# Autodesk Inventor assembly: partial assembly
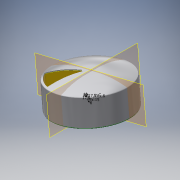
[picture p0: Inventor's stored thumbnail of the model, 180x180]
Saved by Autodesk Inventor 2019 (Build 230136000, 136)
## iProperties
Created: 2019-04-05
Part Number: partial assembly
Document SubType Name: Assembly
Designer: jmc
Author: jmc
## Documents named in this file (7)
- C:\Users\l0086\Desktop\Models\CatFeeder\Case\version6\partial assembly.iam
- C:\Users\l0086\Desktop\Models\CatFeeder\Case\version6\wheel8.ipt
- C:\Users\l0086\Desktop\Models\CatFeeder\Case\version6\Cover.ipt
- C:\Users\l0086\Desktop\Models\3party\Stepper\Stepper 28BYJ48.ipt
- C:\Users\l0086\Desktop\Models\3party\Stepper\ULN2003 Stepper Driver\ULN2003 Stepper Driver.iam
- C:\Users\l0086\Desktop\Models\3party\ESP32\ESP-32_v1.iam
- C:\Users\l0086\Desktop\Models\3party\battery holder\User Library-R6_AA_UM3-1_5V_holder4AA.ipt
## Components (6 placed, 6 different names)
1. wheel8:1 — Rigid:1, Rotational:1, Rotational:2, Rotational:3
2. Cover:1
3. Stepper 28BYJ48:1 — Rigid:1
4. ULN2003 Stepper Driver:1 [sub-assembly] — Rotational:3
5. ESP-32_v1:1 [sub-assembly] — Rotational:2
6. User Library-R6_AA_UM3-1_5V_holder4AA:1 — Rotational:1
## Relationships (4: RevoluteJoint 3, WeldJoint 1)
- Rigid:1 [WeldJoint]: wheel8:1 ↔ Stepper 28BYJ48:1
- Rotational:1 [RevoluteJoint]: wheel8:1 ↔ User Library-R6_AA_UM3-1_5V_holder4AA:1
- Rotational:2 [RevoluteJoint]: wheel8:1 ↔ ESP-32_v1:1
- Rotational:3 [RevoluteJoint]: wheel8:1 ↔ ULN2003 Stepper Driver:1
